# Autodesk Inventor assembly: gearbox4_000_Assembly
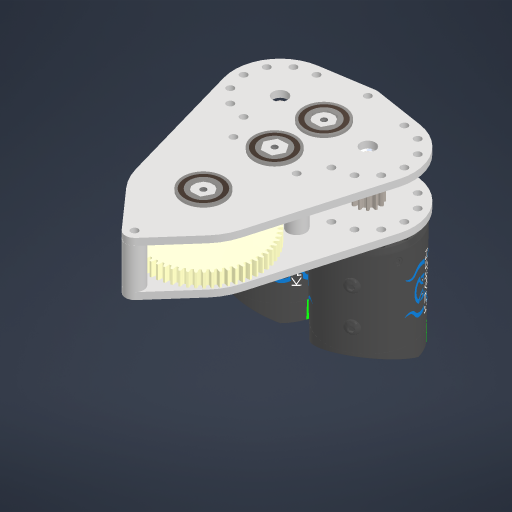
[picture p0: Inventor's stored thumbnail of the model, 512x512]
Saved by Autodesk Inventor 2024.4 (Build 284460000, 460)
## iProperties
Created: 2026-06-12
Part Number: gearbox4_000_Assembly
Document SubType Name: Assembly
Designer: stanr
Author: stanr
## Documents named in this file (10)
- C:\Users\stanr\Documents\GitHub\2026-2027-DesignTraining\Stan\Gearbox4\gearbox4_000_Assembly.iam
- C:\Users\stanr\Documents\GitHub\2026-2027-DesignTraining\Stan\Gearbox4\Gearbox4_001_Plate.ipt
- C:\Users\stanr\Documents\GitHub\2026-2027-DesignTraining\Stan\Gearbox4\WCP-1010\WCP-1010\WCP-1010.ipt
- C:\Users\stanr\Documents\GitHub\2026-2027-DesignTraining\COTS Library\Motors\COTS_WCP-0940_KrakenX60_New.ipt
- C:\Users\stanr\Documents\GitHub\2026-2027-DesignTraining\COTS Library\Motion\Bearings\COTS_WCP-0783_1.125ODHexBearing.ipt
- C:\Users\stanr\Documents\GitHub\2026-2027-DesignTraining\COTS Library\Motion\Gears\20DP gears\Aluminum\COTS_WCP-0720_60T_0.5inHex.ipt
- C:\Users\stanr\Documents\GitHub\2026-2027-DesignTraining\Stan\Gearbox4\WCP-0709\WCP-0709\WCP-0709.ipt
- C:\Users\stanr\Documents\GitHub\2026-2027-DesignTraining\COTS Library\Motion\Gears\20DP gears\Aluminum\COTS_WCP-0700_18T_0.5inHex.ipt
- C:\Users\stanr\Documents\GitHub\2026-2027-DesignTraining\Stan\Gearbox4\Gearbox4_002_Standoff.ipt
- C:\Users\stanr\Documents\GitHub\2026-2027-DesignTraining\Stan\Gearbox4\Gearbox4_003_Hexshaft.ipt
## Components (22 placed, 9 different names)
1. Gearbox4_001_Plate:1 — Mate:32, Mate:33, Mate:34, Mate:41, Mate:42, Mate:43, Mate:44, Mate:45, Mate:46
2. Gearbox4_001_Plate:2 — Mate:1, Mate:3, Mate:4, Mate:5, Mate:6, Mate:7, Mate:10, Mate:11, Mate:12, Mate:13, Mate:14, Mate:15, Mate:16, Mate:17, Mate:24, Mate:25, Mate:26, Mate:27, Mate:28, Mate:29, Mate:30, Mate:31
3. WCP-1010:1 — Mate:9, Mate:10
4. WCP-1010:2 — Mate:8, Mate:11
5. COTS_WCP-0940_KrakenX60_New:1 — Mate:4, Mate:5, Mate:6, Mate:9
6. COTS_WCP-0940_KrakenX60_New:2 — Mate:1, Mate:3, Mate:7, Mate:8
7. COTS_WCP-0783_1.125ODHexBearing:1 — Mate:14, Mate:17, Mate:21, Mate:22, Mate:36, Mate:40
8. COTS_WCP-0783_1.125ODHexBearing:2 — Mate:13, Mate:16, Mate:18, Mate:23, Mate:35, Mate:39
9. COTS_WCP-0783_1.125ODHexBearing:3 — Mate:12, Mate:15, Mate:19, Mate:20, Mate:37, Mate:38
10. COTS_WCP-0720_60T_0.5inHex:1 — Mate:21, Mate:22
11. WCP-0709:1 — Mate:19, Mate:20
12. COTS_WCP-0700_18T_0.5inHex:1 — Mate:18, Mate:23
13. Gearbox4_002_Standoff:1 — Mate:26, Mate:30
14. Gearbox4_002_Standoff:2 — Mate:25, Mate:31
15. Gearbox4_002_Standoff:3 — Mate:27, Mate:28, Mate:32
16. Gearbox4_002_Standoff:4 — Mate:24, Mate:29, Mate:33, Mate:34
17. Gearbox4_003_Hexshaft:1 — Mate:36, Mate:40
18. Gearbox4_003_Hexshaft:2 — Mate:35, Mate:39
19. Gearbox4_003_Hexshaft:3 — Mate:37, Mate:38
20. COTS_WCP-0783_1.125ODHexBearing:4 — Mate:43, Mate:44
21. COTS_WCP-0783_1.125ODHexBearing:5 — Mate:42, Mate:46
22. COTS_WCP-0783_1.125ODHexBearing:6 — Mate:41, Mate:45
## Relationships (45: Mate 45)
- Mate:1: Gearbox4_001_Plate:2 ↔ COTS_WCP-0940_KrakenX60_New:2
- Mate:3: Gearbox4_001_Plate:2 ↔ COTS_WCP-0940_KrakenX60_New:2
- Mate:4: Gearbox4_001_Plate:2 ↔ COTS_WCP-0940_KrakenX60_New:1
- Mate:5: Gearbox4_001_Plate:2 ↔ COTS_WCP-0940_KrakenX60_New:1
- Mate:6: Gearbox4_001_Plate:2 ↔ COTS_WCP-0940_KrakenX60_New:1
- Mate:7: Gearbox4_001_Plate:2 ↔ COTS_WCP-0940_KrakenX60_New:2
- Mate:8: WCP-1010:2 ↔ COTS_WCP-0940_KrakenX60_New:2
- Mate:9: WCP-1010:1 ↔ COTS_WCP-0940_KrakenX60_New:1
- Mate:10: Gearbox4_001_Plate:2 ↔ WCP-1010:1
- Mate:11: Gearbox4_001_Plate:2 ↔ WCP-1010:2
- Mate:12: Gearbox4_001_Plate:2 ↔ COTS_WCP-0783_1.125ODHexBearing:3
- Mate:13: Gearbox4_001_Plate:2 ↔ COTS_WCP-0783_1.125ODHexBearing:2
- Mate:14: Gearbox4_001_Plate:2 ↔ COTS_WCP-0783_1.125ODHexBearing:1
- Mate:15: Gearbox4_001_Plate:2 ↔ COTS_WCP-0783_1.125ODHexBearing:3
- Mate:16: Gearbox4_001_Plate:2 ↔ COTS_WCP-0783_1.125ODHexBearing:2
- Mate:17: Gearbox4_001_Plate:2 ↔ COTS_WCP-0783_1.125ODHexBearing:1
- Mate:18: COTS_WCP-0783_1.125ODHexBearing:2 ↔ COTS_WCP-0700_18T_0.5inHex:1
- Mate:19: COTS_WCP-0783_1.125ODHexBearing:3 ↔ WCP-0709:1
- Mate:20: COTS_WCP-0783_1.125ODHexBearing:3 ↔ WCP-0709:1
- Mate:21: COTS_WCP-0783_1.125ODHexBearing:1 ↔ COTS_WCP-0720_60T_0.5inHex:1
- Mate:22: COTS_WCP-0783_1.125ODHexBearing:1 ↔ COTS_WCP-0720_60T_0.5inHex:1
- Mate:23: COTS_WCP-0783_1.125ODHexBearing:2 ↔ COTS_WCP-0700_18T_0.5inHex:1
- Mate:24: Gearbox4_001_Plate:2 ↔ Gearbox4_002_Standoff:4
- Mate:25: Gearbox4_001_Plate:2 ↔ Gearbox4_002_Standoff:2
- Mate:26: Gearbox4_001_Plate:2 ↔ Gearbox4_002_Standoff:1
- Mate:27: Gearbox4_001_Plate:2 ↔ Gearbox4_002_Standoff:3
- Mate:28: Gearbox4_001_Plate:2 ↔ Gearbox4_002_Standoff:3
- Mate:29: Gearbox4_001_Plate:2 ↔ Gearbox4_002_Standoff:4
- Mate:30: Gearbox4_001_Plate:2 ↔ Gearbox4_002_Standoff:1
- Mate:31: Gearbox4_001_Plate:2 ↔ Gearbox4_002_Standoff:2
- Mate:32: Gearbox4_001_Plate:1 ↔ Gearbox4_002_Standoff:3
- Mate:33: Gearbox4_001_Plate:1 ↔ Gearbox4_002_Standoff:4
- Mate:34: Gearbox4_001_Plate:1 ↔ Gearbox4_002_Standoff:4
- Mate:35: COTS_WCP-0783_1.125ODHexBearing:2 ↔ Gearbox4_003_Hexshaft:2
- Mate:36: COTS_WCP-0783_1.125ODHexBearing:1 ↔ Gearbox4_003_Hexshaft:1
- Mate:37: COTS_WCP-0783_1.125ODHexBearing:3 ↔ Gearbox4_003_Hexshaft:3
- Mate:38: COTS_WCP-0783_1.125ODHexBearing:3 ↔ Gearbox4_003_Hexshaft:3
- Mate:39: COTS_WCP-0783_1.125ODHexBearing:2 ↔ Gearbox4_003_Hexshaft:2
- Mate:40: COTS_WCP-0783_1.125ODHexBearing:1 ↔ Gearbox4_003_Hexshaft:1
- Mate:41: Gearbox4_001_Plate:1 ↔ COTS_WCP-0783_1.125ODHexBearing:6
- Mate:42: Gearbox4_001_Plate:1 ↔ COTS_WCP-0783_1.125ODHexBearing:5
- Mate:43: Gearbox4_001_Plate:1 ↔ COTS_WCP-0783_1.125ODHexBearing:4
- Mate:44: Gearbox4_001_Plate:1 ↔ COTS_WCP-0783_1.125ODHexBearing:4
- Mate:45: Gearbox4_001_Plate:1 ↔ COTS_WCP-0783_1.125ODHexBearing:6
- Mate:46: Gearbox4_001_Plate:1 ↔ COTS_WCP-0783_1.125ODHexBearing:5
